# Autodesk Inventor assembly: assembly endstop
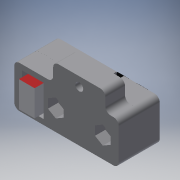
[picture p0: Inventor's stored thumbnail of the model, 180x180]
Saved by Autodesk Inventor 2016 SP1 (Build 200210100, 210)
## iProperties
Created: 2016-04-16
Part Number: assembly endstop
Document SubType Name: Assembly
Designer: ubik
Author: ubik
## Documents named in this file (4)
- E:\GitHub\kossel-XXL\assembly endstop.iam
- E:\GitHub\kossel-XXL\optical endstop.ipt
- E:\GitHub\kossel-XXL\optical endstop base.ipt
- E:\GitHub\kossel-XXL\optical endstop top.ipt
## Components (3 placed, 3 different names)
1. optical endstop:1 — Flush:1
2. optical endstop base:1 — Flush:1, Flush:2, Flush:3
3. optical endstop top:1 — Flush:2, Flush:3
## Relationships (3: Flush 3)
- Flush:1: optical endstop:1 ↔ optical endstop base:1
- Flush:2: optical endstop base:1 ↔ optical endstop top:1
- Flush:3: optical endstop base:1 ↔ optical endstop top:1
